# Autodesk Inventor assembly: Assembly4
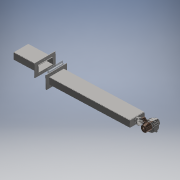
[picture p0: Inventor's stored thumbnail of the model, 180x180]
Saved by Autodesk Inventor 2017 (Build 210142000, 142)
## iProperties
Created: 2017-03-22
Part Number: Assembly4
Document SubType Name: Assembly
Designer: XuZhiqing
Author: XuZhiqing
## Documents named in this file (4)
- C:\Users\XuZhiqing\Desktop\Project01-APS490-CAD-CFD2\CAD-Whole Sys Final2\ZSYSTEM1\Assembly4.iam
- C:\Users\XuZhiqing\Desktop\Project01-APS490-CAD-CFD2\CAD-Whole Sys Final2\ZSYSTEM1\2059K120_DC BLOWER.ipt
- C:\Users\XuZhiqing\Desktop\Project01-APS490-CAD-CFD2\CAD-Whole Sys Final2\ZSYSTEM1\filter.iam
- C:\Users\XuZhiqing\Desktop\Project01-APS490-CAD-CFD2\CAD-Whole Sys Final2\filter and gauge\filter\Part1.ipt
## Components (3 placed, 3 different names)
1. 2059K120_DC BLOWER:1 — Mate:1, Angle:1
2. filter:1 [sub-assembly] — Mate:1, Angle:1, Angle:2, Flush:1, Flush:2
3. Part1:1 — Angle:2, Flush:1, Flush:2
## Relationships (5: Angle 2, Flush 2, Mate 1)
- Mate:1: 2059K120_DC BLOWER:1 ↔ filter:1
- Angle:1 (0 deg): 2059K120_DC BLOWER:1 ↔ filter:1
- Angle:2 (0 deg): filter:1 ↔ Part1:1
- Flush:1: filter:1 ↔ Part1:1
- Flush:2: filter:1 ↔ Part1:1
